# Autodesk Inventor assembly: Ball Valve Actuator
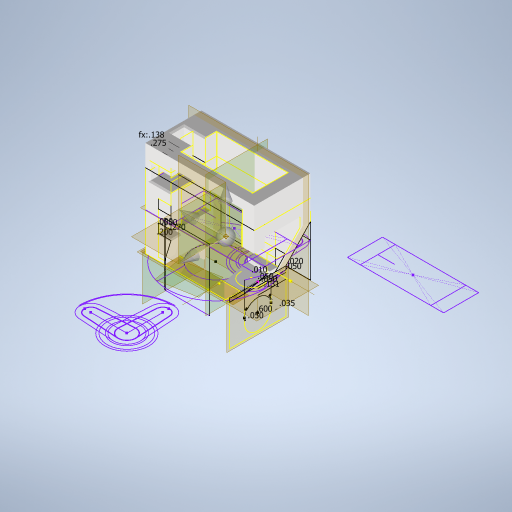
[picture p0: Inventor's stored thumbnail of the model, 512x512]
Saved by Autodesk Inventor 2024 (Build 280153000, 153)
## iProperties
Created: 2024-11-25
Part Number: Ball Valve Actuator
Document SubType Name: Assembly
Designer: Tommy Rohmann
Author: Tommy Rohmann
## Documents named in this file (4)
- C:\Users\Tommy Rohmann\OneDrive\Projects\Microgravity-Press-Washing-Machine\System Design and Documentation\Inventor Design Project\Actuated Ball Valves\V6\Ball Valve Actuator.iam
- C:\Users\Tommy Rohmann\OneDrive\Projects\Microgravity-Press-Washing-Machine\System Design and Documentation\Inventor Design Project\Actuated Ball Valves\V6\Ball Valve Mount.ipt
- C:\Users\Tommy Rohmann\OneDrive\Projects\Microgravity-Press-Washing-Machine\System Design and Documentation\Inventor Design Project\Actuated Ball Valves\V6\Servo Adapter.ipt
- C:\Users\Tommy Rohmann\OneDrive\Projects\Microgravity-Press-Washing-Machine\System Design and Documentation\Inventor Design Project\Actuated Ball Valves\V6\Servo Mount.ipt
## Components (3 placed, 3 different names)
1. Ball Valve Mount:1 — Mate:1, Mate:2, Flush:1, Flush:2, Flush:3, Flush:4
2. Servo Adapter:1 — Mate:1, Mate:2
3. Servo Mount:1 — Flush:1, Flush:2, Flush:3, Flush:4
## Relationships (6: Flush 4, Mate 2)
- Mate:1: Ball Valve Mount:1 ↔ Servo Adapter:1
- Mate:2: Ball Valve Mount:1 ↔ Servo Adapter:1
- Flush:1: Ball Valve Mount:1 ↔ Servo Mount:1
- Flush:2: Ball Valve Mount:1 ↔ Servo Mount:1
- Flush:3 (21.463 mm): Ball Valve Mount:1 ↔ Servo Mount:1
- Flush:4: Ball Valve Mount:1 ↔ Servo Mount:1
